# Autodesk Inventor assembly: jst-ph-5p
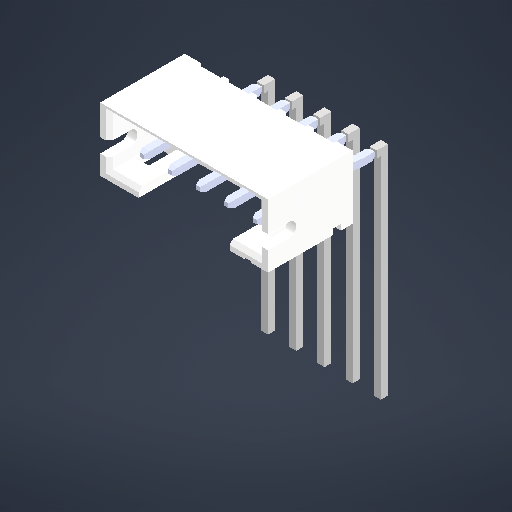
[picture p0: Inventor's stored thumbnail of the model, 512x512]
Saved by Autodesk Inventor 2025.2 (Build 292293000, 293)
## iProperties
Created: 2025-12-13
Part Number: jst-ph-5p
Document SubType Name: Assembly
Designer: sam
Author: sam
## iProperties of the stored document B5B-PH-K-S(LF)(SN).ipt
Created: 2025-12-13
Part Number: B5B-PH-K-S(LF)(SN)
Material: Generic
Document SubType Name: Modeling
Designer: sam
Density: 1 g/cm^3
Appearance: Default
Author: sam
Revision Number: ANY
## iProperties of the stored document B5B-PH-K-S.iam
Created: 2021-10-17
Part Number: B5B-PH-K-S
Description: STEP AP214
Document SubType Name: Assembly
Designer: sam
Sending System: SolidWorks 2017
Preprocessor: SwSTEP 2.0
Title: B5B-PH-K-S(LF)(SN).STEP
Revision Number: ANY
## Documents named in this file (6)
- G:\projects\primary\regulated-irrigation-system\model\asm\electronic-components\jst-ph-5p\jst-ph-5p.iam
- **G:\projects\primary\regulated-irrigation-system\model\asm\electronic-components\jst-ph-5p\jst-ph-5p.iam*LocalDocs*xAaaaqrdaAaaaaaaaAaaaqzvoDh*B5B-PH-K-S.iam
- G:\projects\primary\regulated-irrigation-system\model\asm\electronic-components\jst-ph-5p\jst-ph-5p_wire.ipt
- **G:\projects\primary\regulated-irrigation-system\model\asm\pcb\jst-ph-5p\jst-ph-5p.iam*LocalDocs*xAaaaaydaAaaaaaaaAaaaqqhwDd*B5B-PH-K-S(LF)(SN).ipt
- **G:\projects\primary\regulated-irrigation-system\model\asm\pcb\jst-ph-5p\jst-ph-5p.iam*LocalDocs*xAaaaqrdaAaaaaaaaAaaaqzvoDh*B5B-PH-K-S.iam
- G:\docs\kicad-libraries\B5B-PH-K-S\B5B-PH-K-S.step
## Components (6 placed, 2 different names)
1. B5B-PH-K-S:1 [sub-assembly] — Mate:2, Mate:3, Mate:4, Mate:5, Mate:6, Flush:1, Flush:2, Flush:3, Flush:4, Flush:5, Flush:6, Flush:7, Flush:8, Flush:9, Flush:10
2. jst-ph-5p_wire:1 — Mate:2, Flush:1, Flush:6
3. jst-ph-5p_wire:2 — Mate:3, Flush:2, Flush:7
4. jst-ph-5p_wire:3 — Mate:4, Flush:3, Flush:8
5. jst-ph-5p_wire:4 — Mate:5, Flush:4, Flush:9
6. jst-ph-5p_wire:5 — Mate:6, Flush:5, Flush:10
## Relationships (15: Flush 10, Mate 5)
- Mate:2: B5B-PH-K-S:1 ↔ jst-ph-5p_wire:1
- Mate:3: B5B-PH-K-S:1 ↔ jst-ph-5p_wire:2
- Mate:4: B5B-PH-K-S:1 ↔ jst-ph-5p_wire:3
- Mate:5: B5B-PH-K-S:1 ↔ jst-ph-5p_wire:4
- Mate:6: B5B-PH-K-S:1 ↔ jst-ph-5p_wire:5
- Flush:1: B5B-PH-K-S:1 ↔ jst-ph-5p_wire:1
- Flush:2: B5B-PH-K-S:1 ↔ jst-ph-5p_wire:2
- Flush:3: B5B-PH-K-S:1 ↔ jst-ph-5p_wire:3
- Flush:4: B5B-PH-K-S:1 ↔ jst-ph-5p_wire:4
- Flush:5: B5B-PH-K-S:1 ↔ jst-ph-5p_wire:5
- Flush:6: B5B-PH-K-S:1 ↔ jst-ph-5p_wire:1
- Flush:7: B5B-PH-K-S:1 ↔ jst-ph-5p_wire:2
- Flush:8: B5B-PH-K-S:1 ↔ jst-ph-5p_wire:3
- Flush:9: B5B-PH-K-S:1 ↔ jst-ph-5p_wire:4
- Flush:10: B5B-PH-K-S:1 ↔ jst-ph-5p_wire:5
